# Autodesk Inventor assembly: сборка микроконтроллера
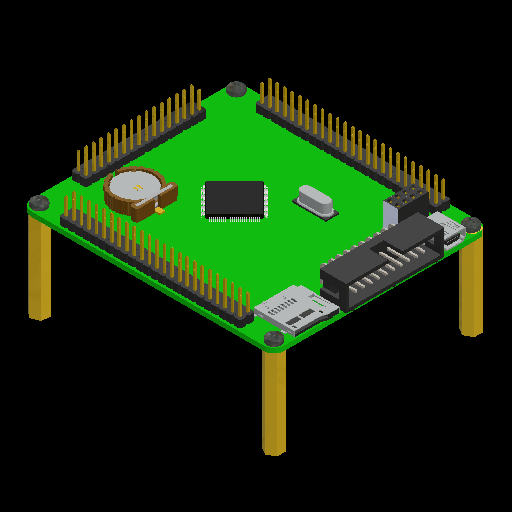
[picture p0: Inventor's stored thumbnail of the model, 512x512]
Saved by Autodesk Inventor 2025 (Build 290162000, 162)
## iProperties
Created: 2025-03-03
Part Number: сборка микроконтроллера
Document SubType Name: Assembly
Designer: volko
Mass: 38.0188 g
Surface Area: 300.785 cm^2
Volume: 18.0259 cm^3
Density: 2.10912 g/cm^3
Author: volko
## Documents named in this file (4)
- C:\Users\volko\Desktop\диплом\Модели\детали\сборка микроконтроллера.iam
- C:\Users\volko\Desktop\диплом\Модели\детали\втулки крепления электроники.ipt
- C:\Users\volko\Desktop\диплом\Модели\детали\stm32.ipt
- C:\Users\volko\Desktop\диплом\Модели\детали\стандартные изделия\ru-RU\ISO 7045  H\ISO 7045 - M2,5 x 8_ - 4.8 - H - ISO.ipt
## Components (9 placed, 3 different names)
1. втулки крепления электроники:1 — Совмещение:3, Совмещение:6, Совмещение:9
2. втулки крепления электроники:2 — Совмещение:2, Совмещение:5
3. втулки крепления электроники:3 — Совмещение:7, Совмещение:8
4. втулки крепления электроники:4 — Совмещение:1, Совмещение:4
5. stm32:1 — Совмещение:1, Совмещение:2, Совмещение:3, Совмещение:4, Совмещение:5, Совмещение:6, Совмещение:7, Совмещение:8, Заподлицо:1, Заподлицо:2, Заподлицо:3, Совмещение:10
6. ISO 7045 H M2,5 x 8 - 4.8 - H:1 — Совмещение:9, Совмещение:10
7. ISO 7045 H M2,5 x 8 - 4.8 - H:2
8. ISO 7045 H M2,5 x 8 - 4.8 - H:3
9. ISO 7045 H M2,5 x 8 - 4.8 - H:4
## Relationships (13: Mate 10, Flush 3)
- Совмещение:1 [Mate]: втулки крепления электроники:4 ↔ stm32:1
- Совмещение:2 [Mate]: втулки крепления электроники:2 ↔ stm32:1
- Совмещение:3 [Mate]: втулки крепления электроники:1 ↔ stm32:1
- Совмещение:4 [Mate]: втулки крепления электроники:4 ↔ stm32:1
- Совмещение:5 [Mate]: втулки крепления электроники:2 ↔ stm32:1
- Совмещение:6 [Mate]: втулки крепления электроники:1 ↔ stm32:1
- Совмещение:7 [Mate]: втулки крепления электроники:3 ↔ stm32:1
- Совмещение:8 [Mate]: втулки крепления электроники:3 ↔ stm32:1
- Заподлицо:1 [Flush]: stm32:1
- Заподлицо:2 [Flush]: stm32:1
- Заподлицо:3 [Flush]: stm32:1
- Совмещение:9 [Mate]: втулки крепления электроники:1 ↔ ISO 7045 H M2,5 x 8 - 4.8 - H:1
- Совмещение:10 [Mate]: stm32:1 ↔ ISO 7045 H M2,5 x 8 - 4.8 - H:1
